# Autodesk Inventor assembly: TB_Fullassemb
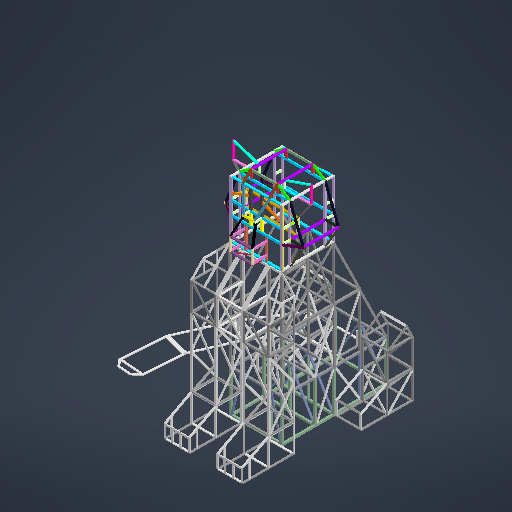
[picture p0: Inventor's stored thumbnail of the model, 512x512]
Saved by Autodesk Inventor 2027.1 (Build 311270010, 270A)
## iProperties
Created: 2025-08-28
Part Number: TB_Fullassemb
Document SubType Name: Assembly
Designer: trott
Author: trott
## Documents named in this file (15)
- C:\Users\jorda\OneDrive\Documents\GitHub\USC-ASME-TigerBurn-2026\CAD\Assembly\TB_Fullassemb.iam
- C:\Users\jorda\OneDrive\Documents\GitHub\USC-ASME-TigerBurn-2026\CAD\Body\Base 01\Base 01.iam
- C:\Users\jorda\OneDrive\Documents\GitHub\USC-ASME-TigerBurn-2026\CAD\Body\Base 02\Base 02.iam
- C:\Users\jorda\OneDrive\Documents\GitHub\USC-ASME-TigerBurn-2026\CAD\Body\Base 03\Base 03.iam
- C:\Users\jorda\OneDrive\Documents\GitHub\USC-ASME-TigerBurn-2026\CAD\Legs\Shoulder\Shoulder_L\Shoulder_L.iam
- C:\Users\jorda\OneDrive\Documents\GitHub\USC-ASME-TigerBurn-2026\CAD\Legs\Shoulder\Shoulder_R\Shoulder_R.iam
- C:\Users\jorda\OneDrive\Documents\GitHub\USC-ASME-TigerBurn-2026\CAD\Legs\Back Leg\B_Leg.iam
- C:\Users\jorda\OneDrive\Documents\GitHub\USC-ASME-TigerBurn-2026\CAD\Legs\Front Leg\F_Leg.iam
- C:\Users\jorda\OneDrive\Documents\GitHub\USC-ASME-TigerBurn-2026\CAD\Legs\Back Foot\B_Foot_v2.iam
- C:\Users\jorda\OneDrive\Documents\GitHub\USC-ASME-TigerBurn-2026\CAD\Legs\Front Foot\F_Foot_v2.iam
- C:\Users\jorda\OneDrive\Documents\GitHub\USC-ASME-TigerBurn-2026\CAD\Tail\tail_p1.iam
- C:\Users\jorda\OneDrive\Documents\GitHub\USC-ASME-TigerBurn-2026\CAD\Tail\tail_p2.iam
- C:\Users\jorda\OneDrive\Documents\GitHub\USC-ASME-TigerBurn-2026\CAD\Tail\tail_p3.iam
- C:\Users\jorda\OneDrive\Documents\GitHub\USC-ASME-TigerBurn-2026\CAD\Tail\tail_p4.iam
- C:\Users\jorda\OneDrive\Documents\GitHub\USC-ASME-TigerBurn-2026\head files\2026 Tiger Burn Head updated 9-4.iam
## Components (18 placed, 14 different names)
1. Base 01:1 [sub-assembly] — Mate:1, Flush:1, Flush:2, Flush:34, Flush:35, Mate:26, Flush:38, Flush:39, Mate:28, Flush:43, Flush:47
2. Base 02:1 [sub-assembly] — Mate:1, Flush:1, Flush:2, Mate:2, Flush:3, Flush:4, Mate:21, Mate:23
3. Base 03:1 [sub-assembly] — Mate:2, Flush:3, Flush:4, Flush:5, Flush:6, Mate:3, Mate:4, Flush:7, Mate:10, Flush:14, Mate:11, Mate:12, Mate:13, Mate:14, Flush:15, Mate:37, Flush:52, Flush:53
4. Shoulder_L:1 [sub-assembly] — Flush:5, Flush:6, Mate:3, Mate:10, Flush:14, Mate:11, Mate:20, Flush:26
5. Shoulder_R:1 [sub-assembly] — Mate:4, Flush:7, Mate:12, Mate:13, Mate:14, Flush:15, Mate:22, Flush:27
6. B_Leg:1 [sub-assembly] — Flush:40, Flush:41, Mate:29
7. B_Leg:2 [sub-assembly] — Flush:36, Flush:37, Mate:27
8. F_Leg:3 [sub-assembly] — Mate:20, Mate:21, Flush:26, Flush:45, Flush:46
9. F_Leg:4 [sub-assembly] — Mate:22, Mate:23, Flush:27, Flush:42, Flush:44
10. B_Foot_v2:1 [sub-assembly] — Flush:34, Flush:35, Mate:26, Flush:36, Flush:37, Mate:27
11. B_Foot_v2:2 [sub-assembly] — Flush:38, Flush:39, Mate:28, Flush:40, Flush:41, Mate:29, Mate:30, Flush:48
12. F_Foot_v2:1 [sub-assembly] — Flush:42, Flush:43, Flush:44
13. F_Foot_v2:2 [sub-assembly] — Flush:45, Flush:46, Flush:47
14. tail_p1:1 [sub-assembly] — Mate:30, Flush:48, Mate:31, Flush:49, Mate:32
15. tail_p2:1 [sub-assembly] — Mate:31, Flush:49, Mate:32, Mate:33, Mate:34, Flush:50
16. tail_p3:1 [sub-assembly] — Mate:33, Mate:34, Flush:50, Mate:35, Flush:51, Mate:36
17. tail_p4:1 [sub-assembly] — Mate:35, Flush:51, Mate:36
18. 2026 Tiger Burn Head updated 9-4:1 [sub-assembly] — Mate:37, Flush:52, Flush:53
## Relationships (56: Flush 31, Mate 25)
- Mate:1: Base 01:1 ↔ Base 02:1
- Flush:1: Base 01:1 ↔ Base 02:1
- Flush:2: Base 01:1 ↔ Base 02:1
- Mate:2: Base 02:1 ↔ Base 03:1
- Flush:3: Base 02:1 ↔ Base 03:1
- Flush:4: Base 02:1 ↔ Base 03:1
- Flush:5: Base 03:1 ↔ Shoulder_L:1
- Flush:6: Base 03:1 ↔ Shoulder_L:1
- Mate:3: Base 03:1 ↔ Shoulder_L:1
- Mate:4: Base 03:1 ↔ Shoulder_R:1
- Flush:7: Base 03:1 ↔ Shoulder_R:1
- Mate:10: Base 03:1 ↔ Shoulder_L:1
- Flush:14: Base 03:1 ↔ Shoulder_L:1
- Mate:11: Base 03:1 ↔ Shoulder_L:1
- Mate:12: Base 03:1 ↔ Shoulder_R:1
- Mate:13: Base 03:1 ↔ Shoulder_R:1
- Mate:14: Base 03:1 ↔ Shoulder_R:1
- Flush:15: Base 03:1 ↔ Shoulder_R:1
- Mate:20: Shoulder_L:1 ↔ F_Leg:3
- Mate:21: Base 02:1 ↔ F_Leg:3
- Flush:26: Shoulder_L:1 ↔ F_Leg:3
- Mate:22: Shoulder_R:1 ↔ F_Leg:4
- Mate:23: Base 02:1 ↔ F_Leg:4
- Flush:27: Shoulder_R:1 ↔ F_Leg:4
- Flush:34: Base 01:1 ↔ B_Foot_v2:1
- Flush:35: Base 01:1 ↔ B_Foot_v2:1
- Mate:26: Base 01:1 ↔ B_Foot_v2:1
- Flush:36: B_Leg:2 ↔ B_Foot_v2:1
- Flush:37: B_Leg:2 ↔ B_Foot_v2:1
- Mate:27: B_Leg:2 ↔ B_Foot_v2:1
- Flush:38: Base 01:1 ↔ B_Foot_v2:2
- Flush:39: Base 01:1 ↔ B_Foot_v2:2
- Mate:28: Base 01:1 ↔ B_Foot_v2:2
- Flush:40: B_Leg:1 ↔ B_Foot_v2:2
- Flush:41: B_Leg:1 ↔ B_Foot_v2:2
- Mate:29: B_Leg:1 ↔ B_Foot_v2:2
- Flush:42: F_Leg:4 ↔ F_Foot_v2:1
- Flush:43: Base 01:1 ↔ F_Foot_v2:1
- Flush:44: F_Leg:4 ↔ F_Foot_v2:1
- Flush:45: F_Leg:3 ↔ F_Foot_v2:2
- Flush:46: F_Leg:3 ↔ F_Foot_v2:2
- Flush:47: Base 01:1 ↔ F_Foot_v2:2
- Mate:30: B_Foot_v2:2 ↔ tail_p1:1
- Flush:48: B_Foot_v2:2 ↔ tail_p1:1
- Mate:31: tail_p1:1 ↔ tail_p2:1
- Flush:49: tail_p1:1 ↔ tail_p2:1
- Mate:32: tail_p1:1 ↔ tail_p2:1
- Mate:33: tail_p2:1 ↔ tail_p3:1
- Mate:34: tail_p2:1 ↔ tail_p3:1
- Flush:50: tail_p2:1 ↔ tail_p3:1
- Mate:35: tail_p3:1 ↔ tail_p4:1
- Flush:51: tail_p3:1 ↔ tail_p4:1
- Mate:36: tail_p3:1 ↔ tail_p4:1
- Mate:37: Base 03:1 ↔ 2026 Tiger Burn Head updated 9-4:1
- Flush:52: Base 03:1 ↔ 2026 Tiger Burn Head updated 9-4:1
- Flush:53: Base 03:1 ↔ 2026 Tiger Burn Head updated 9-4:1
